# Autodesk Inventor assembly: ASSY,ROBOT,2026
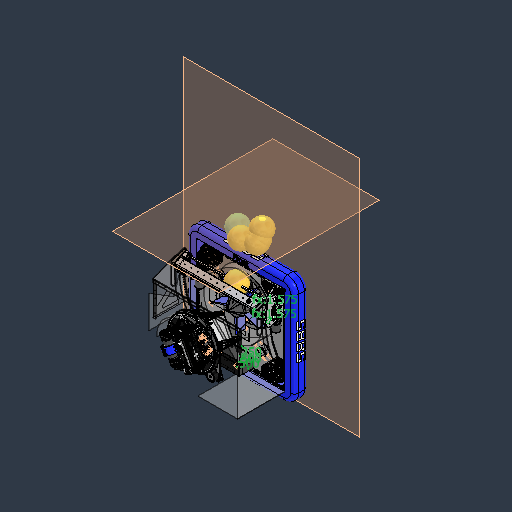
[picture p0: Inventor's stored thumbnail of the model, 512x512]
Saved by Autodesk Inventor 2026 (Build 300175050, 175E)
## iProperties
Created: 2026-01-24
Part Number: ASSY,ROBOT,2026
Document SubType Name: Assembly
Designer: Jthib
Mass: 75094.6 g
Surface Area: 145881 cm^2
Volume: 60890.2 cm^3
Density: 1.23328 g/cm^3
Author: Jthib
## Documents named in this file (17)
- C:\Users\Jthib\Documents\GitHub\2026-Robot-Mechanical\ASSY,ROBOT,2026.iam
- C:\Users\Jthib\Documents\GitHub\2026-Robot-Mechanical\Chassis\CHASSIS.iam
- C:\Users\Jthib\Documents\GitHub\2026-Robot-Mechanical\Spindexer\#Spindexer.iam
- C:\Users\Jthib\Documents\GitHub\2026-Robot-Mechanical\Shooter\Shooter - Front Motors\#SHOOTER.FRONT_MOTORS.iam
- C:\Users\Jthib\Documents\GitHub\2026-Robot-Mechanical\Shooter\Turret\#Turret.iam
- C:\Users\Jthib\Documents\GitHub\2026-Robot-Mechanical\Intake\ASSY,INTAKE.iam
- C:\Users\Jthib\Documents\GitHub\2026-Robot-Mechanical\#2_2026 Field CAD\GE-26900_ Fuel.ipt
- C:\Users\Jthib\Documents\GitHub\2026-Robot-Mechanical\Intake\PLATE,HOPPER,BACK.ipt
- C:\Users\Jthib\Documents\GitHub\2026-Robot-Mechanical\Intake\PLATE,HOPPER,FRONT.ipt
- C:\Users\Jthib\Documents\GitHub\2026-Robot-Mechanical\Intake\PLATE,HOPPER,BACK2.ipt
- C:\Users\Jthib\Documents\GitHub\2026-Robot-Mechanical\#1_CAD Library\Motors\MOTOR,REV,NEO,V1-1.ipt
- C:\Users\Jthib\Documents\GitHub\2026-Robot-Mechanical\Chassis\Bumpers.ipt
- C:\Users\Jthib\Documents\GitHub\2026-Robot-Mechanical\LINEAR_INTAKE\ASSY,INTAKE,LINEAR.iam
- C:\Users\Jthib\Documents\GitHub\2026-Robot-Mechanical\LINEAR_INTAKE\#old-linear-intake\LINEAR_INTAKE_ASSY.iam
- C:\Users\Jthib\Documents\GitHub\2026-Robot-Mechanical\Intake\PURCHASED,20-1,90deg,MAX-PLANETARY.ipt
- C:\Users\Jthib\Documents\GitHub\2026-Robot-Mechanical\LINEAR_INTAKE\MOUNT,KICKER.ipt
- C:\Users\Jthib\Documents\GitHub\2026-Robot-Mechanical\LINEAR_INTAKE\ARM,KICKER.ipt
## Components (19 placed, 16 different names)
1. CHASSIS:1 [sub-assembly] — Flush:1, Flush:2, Flush:3, Mate:9, Mate:10, Mate:11, Tangent:1, Mate:13, Mate:18, Mate:19, Mate:20, Mate:21, Flush:23, Mate:22, Flush:24, Mate:23, Mate:25, Flush:25, Mate:29, Mate:30, Flush:27
2. #Spindexer:1 [sub-assembly] — Mate:11, Mate:12, Tangent:1, Mate:13, Mate:15, Mate:16, Mate:17, Mate:18
3. #SHOOTER.FRONT_MOTORS:1 [sub-assembly] — Mate:9, Mate:10, Mate:12, Insert:1, Mate:14
4. #Turret:1 [sub-assembly] — Insert:1, Mate:14, Mate:15, Mate:16, Mate:17
5. GE-26900_ Fuel:1
6. PLATE,HOPPER,BACK:1 — Flush:23, Mate:22, Flush:24, Mate:24
7. PLATE,HOPPER,FRONT:1 — Mate:23, Mate:24
8. MOTOR,REV,NEO,V1-1:2 — Insert:3
9. Bumpers:1 — Mate:29, Mate:30, Flush:26
10. ASSY,INTAKE,LINEAR:1 [sub-assembly] — Mate:32, Mate:33, Mate:37, Flush:28, Mate:38
11. LINEAR_INTAKE_ASSY:1 [sub-assembly]
12. MOTOR,REV,NEO,V1-1:3
13. PURCHASED,20-1,90deg,MAX-PLANETARY:2 — Mate:32, Mate:33
14. MOUNT,KICKER:1 — Mate:36, Mate:37, Flush:28, Mate:38, Mate:39
15. ARM,KICKER:1 — Mate:36, Mate:39
16. MOTOR,REV,NEO,V1-1:1
17. PURCHASED,20-1,90deg,MAX-PLANETARY:1
18. PLATE,HOPPER,BACK2:1 — Mate:25, Flush:25
19. ASSY,INTAKE:1 [sub-assembly] — Mate:19, Mate:20, Mate:21, Insert:3
## Relationships (44: Mate 29, Flush 9, Insert 5, Tangent 1)
- Flush:1 (-349.25 mm): CHASSIS:1
- Flush:2 (349.25 mm): CHASSIS:1
- Flush:3: CHASSIS:1
- Mate:9 (-190.5 mm): CHASSIS:1 ↔ #SHOOTER.FRONT_MOTORS:1
- Mate:10 (-190.5 mm): CHASSIS:1 ↔ #SHOOTER.FRONT_MOTORS:1
- Mate:11: CHASSIS:1 ↔ #Spindexer:1
- Mate:12 (79.375 mm): #Spindexer:1 ↔ #SHOOTER.FRONT_MOTORS:1
- Tangent:1: CHASSIS:1 ↔ #Spindexer:1
- Mate:13 (-304.8 mm): CHASSIS:1 ↔ #Spindexer:1
- Insert:1: #SHOOTER.FRONT_MOTORS:1 ↔ #Turret:1
- Mate:14: #SHOOTER.FRONT_MOTORS:1 ↔ #Turret:1
- Mate:15: #Spindexer:1 ↔ #Turret:1
- Mate:16: #Spindexer:1 ↔ #Turret:1
- Mate:17: #Spindexer:1 ↔ #Turret:1
- Mate:18: CHASSIS:1 ↔ #Spindexer:1
- Mate:19: CHASSIS:1 ↔ ASSY,INTAKE:1
- Mate:20: CHASSIS:1 ↔ ASSY,INTAKE:1
- Mate:21: CHASSIS:1 ↔ ASSY,INTAKE:1
- Flush:23: CHASSIS:1 ↔ PLATE,HOPPER,BACK:1
- Mate:22: CHASSIS:1 ↔ PLATE,HOPPER,BACK:1
- Flush:24: CHASSIS:1 ↔ PLATE,HOPPER,BACK:1
- Mate:23: CHASSIS:1 ↔ PLATE,HOPPER,FRONT:1
- Mate:24: PLATE,HOPPER,BACK:1 ↔ PLATE,HOPPER,FRONT:1
- Mate:25: CHASSIS:1 ↔ PLATE,HOPPER,BACK2:1
- Flush:25: CHASSIS:1 ↔ PLATE,HOPPER,BACK2:1
- [Insert]: MOTOR,REV,NEO,V1-1:1 ↔ PURCHASED,20-1,90deg,MAX-PLANETARY:1
- Insert:3: MOTOR,REV,NEO,V1-1:2 ↔ ASSY,INTAKE:1
- [Mate]: CHASSIS:1 ↔ ASSY,INTAKE,LINEAR:1
- [Mate]: CHASSIS:1 ↔ ASSY,INTAKE,LINEAR:1
- [Mate]: CHASSIS:1 ↔ ASSY,INTAKE,LINEAR:1
- Mate:29: CHASSIS:1 ↔ Bumpers:1
- Mate:30: CHASSIS:1 ↔ Bumpers:1
- Flush:26 (-165.1 mm): Bumpers:1
- Flush:27 (304.8 mm): CHASSIS:1
- [Insert]: PURCHASED,20-1,90deg,MAX-PLANETARY:1 ↔ ASSY,INTAKE:1
- [Mate]: PURCHASED,20-1,90deg,MAX-PLANETARY:1 ↔ ASSY,INTAKE:1
- [Insert]: MOTOR,REV,NEO,V1-1:3 ↔ PURCHASED,20-1,90deg,MAX-PLANETARY:2
- Mate:32: ASSY,INTAKE,LINEAR:1 ↔ PURCHASED,20-1,90deg,MAX-PLANETARY:2
- Mate:33: ASSY,INTAKE,LINEAR:1 ↔ PURCHASED,20-1,90deg,MAX-PLANETARY:2
- Mate:36: MOUNT,KICKER:1 ↔ ARM,KICKER:1
- Mate:37: ASSY,INTAKE,LINEAR:1 ↔ MOUNT,KICKER:1
- Flush:28: ASSY,INTAKE,LINEAR:1 ↔ MOUNT,KICKER:1
- Mate:38: ASSY,INTAKE,LINEAR:1 ↔ MOUNT,KICKER:1
- Mate:39: MOUNT,KICKER:1 ↔ ARM,KICKER:1
## Named parameters: d105_d89 = 0 mm
